# Autodesk Inventor assembly: Сборка
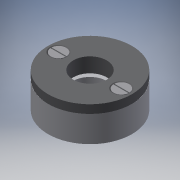
[picture p0: Inventor's stored thumbnail of the model, 180x180]
Saved by Autodesk Inventor 2019.3 (Build 233278000, 278)
## iProperties
Created: 2020-04-02
Part Number: Сборка
Material: Типовые
Document SubType Name: Assembly
Designer: Admin
Mass: 127.434 g
Surface Area: 312.491 cm^2
Volume: 127.434 cm^3
Density: 1 g/cm^3
Author: Admin
## Documents named in this file (5)
- D:\МГТУ Учеба\2 Семестр\Инжграф\Модуль 3\Сборка.iam
- D:\МГТУ Учеба\2 Семестр\Инжграф\Модуль 3\Корпус.ipt
- D:\МГТУ Учеба\2 Семестр\Инжграф\Модуль 3\Крышка.ipt
- C:\Users\Admin\Documents\Inventor\Content Center Files\R2019\ru-RU\GOST 17475-80 (1)\Винт M8-6gx10 ГОСТ 17475-80.ipt
- C:\Users\Admin\Documents\Inventor\Content Center Files\R2019\ru-RU\GOST 17475-80 (1)\Винт M8-6gx16 ГОСТ 17475-80.ipt
## Components (4 placed, 4 different names)
1. Корпус:1 — Совмещение:1, Совмещение:2, Совмещение:3
2. Крышка:1 — Совмещение:1, Совмещение:2, Совмещение:3, Совмещение:4, Совмещение:5
3. Винт ГОСТ 17475-80 M8 x 16:1 — Совмещение:4
4. Винт ГОСТ 17475-80 M8 x 10:1 — Совмещение:5
## Relationships (5: Mate 5)
- Совмещение:1 [Mate]: Корпус:1 ↔ Крышка:1
- Совмещение:2 [Mate]: Корпус:1 ↔ Крышка:1
- Совмещение:3 [Mate]: Корпус:1 ↔ Крышка:1
- Совмещение:4 [Mate]: Крышка:1 ↔ Винт ГОСТ 17475-80 M8 x 16:1
- Совмещение:5 [Mate]: Крышка:1 ↔ Винт ГОСТ 17475-80 M8 x 10:1
